# Autodesk Inventor assembly: ObudowaNowa2
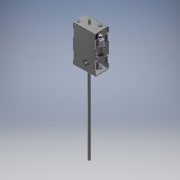
[picture p0: Inventor's stored thumbnail of the model, 180x180]
Saved by Autodesk Inventor 2019 (Build 230136000, 136)
## iProperties
Created: 2020-08-21
Part Number: ObudowaNowa2
Material: Ogólny
Document SubType Name: Assembly
Designer: barto
Author: barto
## Documents named in this file (28)
- C:\Users\estee\OneDrive\Pulpit\estere\1\MUM\wogoleNajnowszyGit\Mechanika\Moduł obrotu RET Estera\prawieKoncowka\ObudowaNowa2.iam
- C:\Users\estee\OneDrive\Pulpit\estere\1\MUM\wogoleNajnowszyGit\Mechanika\Moduł obrotu RET Estera\prawieKoncowka\UCFL-201.ipt
- C:\Users\estee\OneDrive\Pulpit\estere\1\MUM\wogoleNajnowszyGit\Mechanika\Moduł obrotu RET Estera\prawieKoncowka\ModulSilnika.iam
- C:\Users\estee\OneDrive\Pulpit\estere\1\MUM\wogoleNajnowszyGit\Mechanika\Moduł obrotu RET Estera\prawieKoncowka\ModulWalkaNapinajacego.iam
- C:\Users\estee\OneDrive\Pulpit\estere\1\MUM\wogoleNajnowszyGit\Mechanika\Moduł obrotu RET Estera\prawieKoncowka\pasekturbonowy.iam
- C:\Users\estee\OneDrive\Pulpit\estere\1\MUM\wogoleNajnowszyGit\Mechanika\Moduł obrotu RET Estera\prawieKoncowka\DIN 471 - 12 x 1(1).ipt
- C:\Users\estee\OneDrive\Pulpit\estere\1\MUM\wogoleNajnowszyGit\Mechanika\Moduł obrotu RET Estera\prawieKoncowka\uchwytDoNapinacza.ipt
- C:\Users\estee\OneDrive\Pulpit\estere\1\MUM\wogoleNajnowszyGit\Mechanika\Moduł obrotu RET Estera\prawieKoncowka\Połączenie gwintowe1.iam
- C:\Users\estee\OneDrive\Pulpit\estere\1\MUM\wogoleNajnowszyGit\Mechanika\Moduł obrotu RET Estera\prawieKoncowka\Połączenie gwintowe2.iam
- C:\Users\estee\OneDrive\Pulpit\estere\1\MUM\wogoleNajnowszyGit\Mechanika\Moduł obrotu RET Estera\prawieKoncowka\Połączenie gwintowe3.iam
- C:\Users\estee\OneDrive\Pulpit\estere\1\MUM\wogoleNajnowszyGit\Mechanika\Moduł obrotu RET Estera\prawieKoncowka\Połączenie gwintowe4.iam
- C:\Users\estee\OneDrive\Pulpit\estere\1\MUM\wogoleNajnowszyGit\Mechanika\Moduł obrotu RET Estera\prawieKoncowka\Połączenie gwintowe5.iam
- C:\Users\estee\OneDrive\Pulpit\estere\1\MUM\wogoleNajnowszyGit\Mechanika\Moduł obrotu RET Estera\prawieKoncowka\Połączenie gwintowe6.iam
- C:\Users\estee\OneDrive\Pulpit\estere\1\MUM\wogoleNajnowszyGit\Mechanika\Moduł obrotu RET Estera\prawieKoncowka\Połączenie gwintowe7.iam
- C:\Users\estee\OneDrive\Pulpit\estere\1\MUM\wogoleNajnowszyGit\Mechanika\Moduł obrotu RET Estera\prawieKoncowka\Połączenie gwintowe8.iam
- C:\Users\estee\OneDrive\Pulpit\estere\1\MUM\wogoleNajnowszyGit\Mechanika\Moduł obrotu RET Estera\prawieKoncowka\Połączenie gwintowe9.iam
- C:\Users\estee\OneDrive\Pulpit\estere\1\MUM\wogoleNajnowszyGit\Mechanika\Moduł obrotu RET Estera\prawieKoncowka\Połączenie gwintowe10.iam
- C:\Users\estee\OneDrive\Pulpit\estere\1\MUM\wogoleNajnowszyGit\Mechanika\Moduł obrotu RET Estera\prawieKoncowka\ZaslepkaObudowa.ipt
- C:\Users\estee\OneDrive\Pulpit\estere\1\MUM\wogoleNajnowszyGit\Mechanika\Moduł obrotu RET Estera\prawieKoncowka\Połączenie gwintowe11.iam
- C:\Users\estee\OneDrive\Pulpit\estere\1\MUM\wogoleNajnowszyGit\Mechanika\Moduł obrotu RET Estera\prawieKoncowka\Połączenie gwintowe12.iam
- C:\Users\estee\OneDrive\Pulpit\estere\1\MUM\wogoleNajnowszyGit\Mechanika\Moduł obrotu RET Estera\prawieKoncowka\Połączenie gwintowe13.iam
- C:\Users\estee\OneDrive\Pulpit\estere\1\MUM\wogoleNajnowszyGit\Mechanika\Moduł obrotu RET Estera\prawieKoncowka\Połączenie gwintowe14.iam
- C:\Users\estee\OneDrive\Pulpit\estere\1\MUM\wogoleNajnowszyGit\Mechanika\Moduł obrotu RET Estera\prawieKoncowka\GlownaObudowa2.ipt
- C:\Users\estee\OneDrive\Pulpit\estere\1\MUM\wogoleNajnowszyGit\Mechanika\Moduł obrotu RET Estera\prawieKoncowka\kolnierz.ipt
- C:\Users\estee\OneDrive\Pulpit\estere\1\MUM\wogoleNajnowszyGit\Mechanika\Moduł obrotu RET Estera\prawieKoncowka\ISO 7045 - M4 x 5 - 4.8 - H - ISO.ipt
- C:\Users\estee\OneDrive\Pulpit\estere\1\MUM\wogoleNajnowszyGit\Mechanika\Moduł obrotu RET Estera\prawieKoncowka\ModulDuzegoKolaKrotki.iam
- C:\Users\estee\OneDrive\Pulpit\estere\1\MUM\wogoleNajnowszyGit\Mechanika\Moduł obrotu RET Estera\prawieKoncowka\ISO 8676 - M10 x 1 x 20 - ISO.ipt
- C:\Users\estee\OneDrive\Pulpit\estere\1\MUM\wogoleNajnowszyGit\Mechanika\Moduł obrotu RET Estera\prawieKoncowka\ISO 4035 - M10 - ISO.ipt
## Components (48 placed, 14 different names)
1. GlownaObudowa2:1 — Zestawiające:9, Zestawiające:13, Zestawiające:16, Zestawiające:24, Zestawiające:25, Zestawiające:26, Zestawiające:27, Zestawiające:28, Zestawiające:29, Zestawiające:32, Zestawiające:40, Zestawiające:42, Zestawiające:43, Zestawiające:44, Zestawiające:45, Zestawiające:46, Zestawiające:47, Zestawiające:49, Zestawiające:51, Zestawiające:53, Zestawiające:55, Zestawiające:56, Zestawiające:57, Mate:66, Mate:67, Mate:68, Mate:69, Mate:70, Mate:71, Mate:72, Mate:76, Mate:77, Mate:78, Mate:79, Mate:80, Mate:81, Mate:82, Mate:83, Mate:84, Mate:85, Mate:86, Mate:87, Mate:88, Mate:89, Mate:90, Mate:91, Mate:100, Mate:101, Mate:102, Mate:103, Mate:108, Mate:109, Mate:110, Mate:111
2. ModulSilnika:1 [sub-assembly] — Zestawiające:13, Równoległe:1, Zestawiające:12, Zestawiające:16, Zestawiające:48, Zestawiające:50, Zestawiające:52, Zestawiające:54
3. ModulWalkaNapinajacego:1 [sub-assembly] — Zestawiające:15, Zestawiające:33, Zestawiające:34, Zestawiające:35, Styczny:1, Zestawiające:36, Zestawiające:38, Zestawiające:39
4. pasekturbonowy:1 [sub-assembly] — Zestawiające:10, Zestawiające:11, Zestawiające:12, Zestawiające:15, Styczny:1
5. ModulDuzegoKolaKrotki:1 [sub-assembly] — Równoległe:1, Zestawiające:9, Zestawiające:10, Zestawiające:11, Zestawiające:23, Zestawiające:30
6. DIN 471 > 9mm <= 300mm 12 x 1:1 — Zestawiające:23
7. UCFL-201:1 — Zestawiające:24, Zestawiające:25, Zestawiające:26, Mate:104, Mate:106
8. UCFL-201:2 — Zestawiające:27, Zestawiające:28, Zestawiające:29, Zestawiające:31, Mate:112, Mate:114
9. DIN 471 > 9mm <= 300mm 12 x 1:2 — Zestawiające:30, Zestawiające:31
10. uchwytDoNapinacza:1 — Zestawiające:32, Zestawiające:33, Zestawiające:34, Zestawiające:35, Zestawiające:37, Zestawiające:41
11. Połączenie gwintowe:1 [sub-assembly] — Zestawiające:36, Zestawiające:37
12. Połączenie gwintowe:2 [sub-assembly] — Zestawiające:38, Zestawiające:39
13. Połączenie gwintowe:3 [sub-assembly] — Zestawiające:40, Zestawiające:41
14. Połączenie gwintowe:4 [sub-assembly] — Zestawiające:42, Zestawiające:43
15. Połączenie gwintowe:5 [sub-assembly] — Zestawiające:44, Zestawiające:45
16. Połączenie gwintowe:6 [sub-assembly] — Zestawiające:46, Zestawiające:47
17. Połączenie gwintowe:7 [sub-assembly] — Zestawiające:48, Zestawiające:49
18. Połączenie gwintowe:8 [sub-assembly] — Zestawiające:50, Zestawiające:51
19. Połączenie gwintowe:9 [sub-assembly] — Zestawiające:52, Zestawiające:53
20. Połączenie gwintowe:10 [sub-assembly] — Zestawiające:54, Zestawiające:55
21. ZaslepkaObudowa:1 — Zestawiające:56, Zestawiające:57, Zestawiające:58, Zestawiające:59, Zestawiające:60, Zestawiające:61, Zestawiające:62, Zestawiające:63, Zestawiające:64, Zestawiające:65
22. Połączenie gwintowe:11 [sub-assembly] — Zestawiające:58, Zestawiające:59
23. Połączenie gwintowe:12 [sub-assembly] — Zestawiające:60, Zestawiające:61
24. Połączenie gwintowe:13 [sub-assembly] — Zestawiające:62, Zestawiające:63, Mate:88
25. Połączenie gwintowe:14 [sub-assembly] — Zestawiające:64, Zestawiające:65
26. kolnierz:1 — Mate:66, Mate:67, Mate:68, Mate:73, Mate:74, Mate:75
27. kolnierz:2 — Mate:69, Mate:70, Mate:71
28. ISO 7045 H M4 x 5 - 4.8 - H:1 — Mate:74, Mate:79
29. ISO 7045 H M4 x 5 - 4.8 - H:2 — Mate:80, Mate:84
30. ISO 7045 H M4 x 5 - 4.8 - H:3 — Mate:75, Mate:78
31. ISO 7045 H M4 x 5 - 4.8 - H:4 — Mate:73, Mate:76
32. ISO 7045 H M4 x 5 - 4.8 - H:5 — Mate:83, Mate:85
33. ISO 7045 H M4 x 5 - 4.8 - H:6 — Mate:81, Mate:87
34. ISO 7045 H M4 x 5 - 4.8 - H:7 — Mate:82, Mate:86
35. ISO 7045 H M4 x 5 - 4.8 - H:8 — Mate:72, Mate:77
36. ZaslepkaObudowa:2 — Mate:89, Mate:90, Mate:91, Mate:92, Mate:93, Mate:94, Mate:95, Mate:96, Mate:97, Mate:98, Mate:99
37. Połączenie gwintowe:15 [sub-assembly] — Mate:95, Mate:96
38. Połączenie gwintowe:16 [sub-assembly] — Mate:94, Mate:98
39. Połączenie gwintowe:17 [sub-assembly] — Mate:93, Mate:99
40. Połączenie gwintowe:18 [sub-assembly] — Mate:92, Mate:97
41. ISO 8676 M10 x 1 x 20:1 — Mate:100, Mate:102, Mate:105
42. ISO 8676 M10 x 1 x 20:2 — Mate:101, Mate:103, Mate:107
43. ISO 8676 M10 x 1 x 20:3 — Mate:108, Mate:111, Mate:113
44. ISO 8676 M10 x 1 x 20:4 — Mate:109, Mate:110, Mate:115
45. ISO 4035 M10:1 — Mate:106, Mate:107
46. ISO 4035 M10:2 — Mate:104, Mate:105
47. ISO 4035 M10:3 — Mate:112, Mate:113
48. ISO 4035 M10:4 — Mate:114, Mate:115
## Relationships (102: Mate 100, Flush 1, Tangent 1)
- Zestawiające:13 [Mate]: GlownaObudowa2:1 ↔ ModulSilnika:1
- Równoległe:1 [Flush]: ModulSilnika:1 ↔ ModulDuzegoKolaKrotki:1
- Zestawiające:9 [Mate]: GlownaObudowa2:1 ↔ ModulDuzegoKolaKrotki:1
- Zestawiające:10 [Mate] (0.5 mm): pasekturbonowy:1 ↔ ModulDuzegoKolaKrotki:1
- Zestawiające:11 [Mate]: pasekturbonowy:1 ↔ ModulDuzegoKolaKrotki:1
- Zestawiające:12 [Mate]: ModulSilnika:1 ↔ pasekturbonowy:1
- Zestawiające:15 [Mate] (0.5 mm): ModulWalkaNapinajacego:1 ↔ pasekturbonowy:1
- Zestawiające:16 [Mate] (60 mm): GlownaObudowa2:1 ↔ ModulSilnika:1
- Zestawiające:23 [Mate]: ModulDuzegoKolaKrotki:1 ↔ DIN 471 > 9mm <= 300mm 12 x 1:1
- Zestawiające:24 [Mate]: GlownaObudowa2:1 ↔ UCFL-201:1
- Zestawiające:25 [Mate]: GlownaObudowa2:1 ↔ UCFL-201:1
- Zestawiające:26 [Mate]: GlownaObudowa2:1 ↔ UCFL-201:1
- Zestawiające:27 [Mate]: GlownaObudowa2:1 ↔ UCFL-201:2
- Zestawiające:28 [Mate]: GlownaObudowa2:1 ↔ UCFL-201:2
- Zestawiające:29 [Mate]: GlownaObudowa2:1 ↔ UCFL-201:2
- Zestawiające:30 [Mate]: ModulDuzegoKolaKrotki:1 ↔ DIN 471 > 9mm <= 300mm 12 x 1:2
- Zestawiające:31 [Mate]: UCFL-201:2 ↔ DIN 471 > 9mm <= 300mm 12 x 1:2
- Zestawiające:32 [Mate]: GlownaObudowa2:1 ↔ uchwytDoNapinacza:1
- Zestawiające:33 [Mate]: ModulWalkaNapinajacego:1 ↔ uchwytDoNapinacza:1
- Zestawiające:34 [Mate]: ModulWalkaNapinajacego:1 ↔ uchwytDoNapinacza:1
- Zestawiające:35 [Mate]: ModulWalkaNapinajacego:1 ↔ uchwytDoNapinacza:1
- Styczny:1 [Tangent]: ModulWalkaNapinajacego:1 ↔ pasekturbonowy:1
- Zestawiające:36 [Mate]: ModulWalkaNapinajacego:1 ↔ Połączenie gwintowe:1
- Zestawiające:37 [Mate]: uchwytDoNapinacza:1 ↔ Połączenie gwintowe:1
- Zestawiające:38 [Mate]: ModulWalkaNapinajacego:1 ↔ Połączenie gwintowe:2
- Zestawiające:39 [Mate]: ModulWalkaNapinajacego:1 ↔ Połączenie gwintowe:2
- Zestawiające:40 [Mate]: GlownaObudowa2:1 ↔ Połączenie gwintowe:3
- Zestawiające:41 [Mate]: uchwytDoNapinacza:1 ↔ Połączenie gwintowe:3
- Zestawiające:42 [Mate]: GlownaObudowa2:1 ↔ Połączenie gwintowe:4
- Zestawiające:43 [Mate]: GlownaObudowa2:1 ↔ Połączenie gwintowe:4
- Zestawiające:44 [Mate]: GlownaObudowa2:1 ↔ Połączenie gwintowe:5
- Zestawiające:45 [Mate]: GlownaObudowa2:1 ↔ Połączenie gwintowe:5
- Zestawiające:46 [Mate]: GlownaObudowa2:1 ↔ Połączenie gwintowe:6
- Zestawiające:47 [Mate]: GlownaObudowa2:1 ↔ Połączenie gwintowe:6
- Zestawiające:48 [Mate]: ModulSilnika:1 ↔ Połączenie gwintowe:7
- Zestawiające:49 [Mate]: GlownaObudowa2:1 ↔ Połączenie gwintowe:7
- Zestawiające:50 [Mate]: ModulSilnika:1 ↔ Połączenie gwintowe:8
- Zestawiające:51 [Mate]: GlownaObudowa2:1 ↔ Połączenie gwintowe:8
- Zestawiające:52 [Mate]: ModulSilnika:1 ↔ Połączenie gwintowe:9
- Zestawiające:53 [Mate]: GlownaObudowa2:1 ↔ Połączenie gwintowe:9
- Zestawiające:54 [Mate]: ModulSilnika:1 ↔ Połączenie gwintowe:10
- Zestawiające:55 [Mate]: GlownaObudowa2:1 ↔ Połączenie gwintowe:10
- Zestawiające:56 [Mate]: GlownaObudowa2:1 ↔ ZaslepkaObudowa:1
- Zestawiające:57 [Mate]: GlownaObudowa2:1 ↔ ZaslepkaObudowa:1
- Zestawiające:58 [Mate]: ZaslepkaObudowa:1 ↔ Połączenie gwintowe:11
- Zestawiające:59 [Mate]: ZaslepkaObudowa:1 ↔ Połączenie gwintowe:11
- Zestawiające:60 [Mate]: ZaslepkaObudowa:1 ↔ Połączenie gwintowe:12
- Zestawiające:61 [Mate]: ZaslepkaObudowa:1 ↔ Połączenie gwintowe:12
- Zestawiające:62 [Mate]: ZaslepkaObudowa:1 ↔ Połączenie gwintowe:13
- Zestawiające:63 [Mate]: ZaslepkaObudowa:1 ↔ Połączenie gwintowe:13
- Zestawiające:64 [Mate]: ZaslepkaObudowa:1 ↔ Połączenie gwintowe:14
- Zestawiające:65 [Mate]: ZaslepkaObudowa:1 ↔ Połączenie gwintowe:14
- Mate:66: GlownaObudowa2:1 ↔ kolnierz:1
- Mate:67: GlownaObudowa2:1 ↔ kolnierz:1
- Mate:68: GlownaObudowa2:1 ↔ kolnierz:1
- Mate:69: GlownaObudowa2:1 ↔ kolnierz:2
- Mate:70: GlownaObudowa2:1 ↔ kolnierz:2
- Mate:71: GlownaObudowa2:1 ↔ kolnierz:2
- Mate:72: GlownaObudowa2:1 ↔ ISO 7045 H M4 x 5 - 4.8 - H:8
- Mate:73: kolnierz:1 ↔ ISO 7045 H M4 x 5 - 4.8 - H:4
- Mate:74: kolnierz:1 ↔ ISO 7045 H M4 x 5 - 4.8 - H:1
- Mate:75: kolnierz:1 ↔ ISO 7045 H M4 x 5 - 4.8 - H:3
- Mate:76: GlownaObudowa2:1 ↔ ISO 7045 H M4 x 5 - 4.8 - H:4
- Mate:77: GlownaObudowa2:1 ↔ ISO 7045 H M4 x 5 - 4.8 - H:8
- Mate:78: GlownaObudowa2:1 ↔ ISO 7045 H M4 x 5 - 4.8 - H:3
- Mate:79: GlownaObudowa2:1 ↔ ISO 7045 H M4 x 5 - 4.8 - H:1
- Mate:80: GlownaObudowa2:1 ↔ ISO 7045 H M4 x 5 - 4.8 - H:2
- Mate:81: GlownaObudowa2:1 ↔ ISO 7045 H M4 x 5 - 4.8 - H:6
- Mate:82: GlownaObudowa2:1 ↔ ISO 7045 H M4 x 5 - 4.8 - H:7
- Mate:83: GlownaObudowa2:1 ↔ ISO 7045 H M4 x 5 - 4.8 - H:5
- Mate:84: GlownaObudowa2:1 ↔ ISO 7045 H M4 x 5 - 4.8 - H:2
- Mate:85: GlownaObudowa2:1 ↔ ISO 7045 H M4 x 5 - 4.8 - H:5
- Mate:86: GlownaObudowa2:1 ↔ ISO 7045 H M4 x 5 - 4.8 - H:7
- Mate:87: GlownaObudowa2:1 ↔ ISO 7045 H M4 x 5 - 4.8 - H:6
- Mate:88: GlownaObudowa2:1 ↔ Połączenie gwintowe:13
- Mate:89: GlownaObudowa2:1 ↔ ZaslepkaObudowa:2
- Mate:90: GlownaObudowa2:1 ↔ ZaslepkaObudowa:2
- Mate:91: GlownaObudowa2:1 ↔ ZaslepkaObudowa:2
- Mate:92: ZaslepkaObudowa:2 ↔ Połączenie gwintowe:18
- Mate:93: ZaslepkaObudowa:2 ↔ Połączenie gwintowe:17
- Mate:94: ZaslepkaObudowa:2 ↔ Połączenie gwintowe:16
- Mate:95: ZaslepkaObudowa:2 ↔ Połączenie gwintowe:15
- Mate:96: ZaslepkaObudowa:2 ↔ Połączenie gwintowe:15
- Mate:97: ZaslepkaObudowa:2 ↔ Połączenie gwintowe:18
- Mate:98: ZaslepkaObudowa:2 ↔ Połączenie gwintowe:16
- Mate:99: ZaslepkaObudowa:2 ↔ Połączenie gwintowe:17
- Mate:100: GlownaObudowa2:1 ↔ ISO 8676 M10 x 1 x 20:1
- Mate:101: GlownaObudowa2:1 ↔ ISO 8676 M10 x 1 x 20:2
- Mate:102: GlownaObudowa2:1 ↔ ISO 8676 M10 x 1 x 20:1
- Mate:103: GlownaObudowa2:1 ↔ ISO 8676 M10 x 1 x 20:2
- Mate:104: UCFL-201:1 ↔ ISO 4035 M10:2
- Mate:105: ISO 8676 M10 x 1 x 20:1 ↔ ISO 4035 M10:2
- Mate:106: UCFL-201:1 ↔ ISO 4035 M10:1
- Mate:107: ISO 8676 M10 x 1 x 20:2 ↔ ISO 4035 M10:1
- Mate:108: GlownaObudowa2:1 ↔ ISO 8676 M10 x 1 x 20:3
- Mate:109: GlownaObudowa2:1 ↔ ISO 8676 M10 x 1 x 20:4
- Mate:110: GlownaObudowa2:1 ↔ ISO 8676 M10 x 1 x 20:4
- Mate:111: GlownaObudowa2:1 ↔ ISO 8676 M10 x 1 x 20:3
- Mate:112: UCFL-201:2 ↔ ISO 4035 M10:3
- Mate:113: ISO 8676 M10 x 1 x 20:3 ↔ ISO 4035 M10:3
- Mate:114: UCFL-201:2 ↔ ISO 4035 M10:4
- Mate:115: ISO 8676 M10 x 1 x 20:4 ↔ ISO 4035 M10:4
## Named parameters: sa_0 = 10000, sa_1 = 0, sa_2 = 0
note: some values were not read from the file. Shown as the stored number, unit unknown: "sa_0", "sa_1", "sa_2".
